# Autodesk Inventor assembly: Lift.03.01.00.00
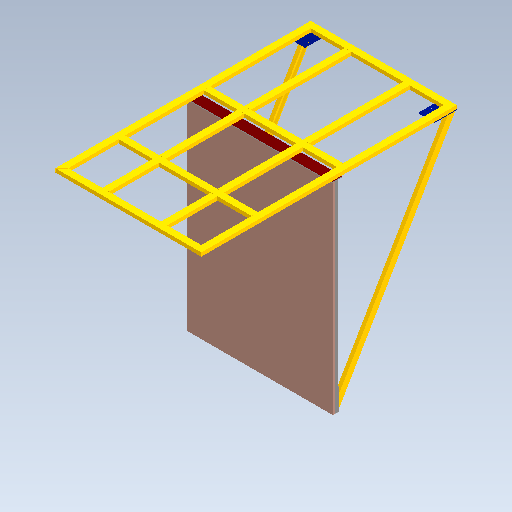
[picture p0: Inventor's stored thumbnail of the model, 512x512]
Saved by Autodesk Inventor 2021 (Build 250183000, 183)
## iProperties
_SolveAssemblyDoc: Frame Generator Solve Assembly
_Version: 15.0.0
Created: 2020-09-20
Part Number: Lift.03.01.00.00
Document SubType Name: Assembly
Designer: Kostya
Author: Kostya
## Documents named in this file (8)
- C:\Lift\Lift.03.01.00.00.iam
- C:\Lift\Lift.03.01.02.00.ipt
- C:\Lift\Lift.03.01.00.00\Frame\Frame 1600622124454.iam
- C:\Lift\Lift.03.01.01.00.iam
- C:\Lift\Lift.03.01.00.03.ipt
- C:\Lift\Lift.03.01.00.02_MIR.ipt
- C:\Lift\Lift.03.01.00.05.ipt
- C:\Lift\Lift.03.01.00.06.ipt
## Components (9 placed, 7 different names)
1. Lift.03.01.02.00:1
2. Frame 1600622124454:1 [sub-assembly] — Заподлицо:4, Заподлицо:5, Заподлицо:6, Заподлицо:7, Заподлицо:8, Совмещение:5, Совмещение:6, Совмещение:7, Заподлицо:12, Совмещение:8, Совмещение:9, Совмещение:10, Заподлицо:15
3. Lift.03.01.01.00:1 [sub-assembly] — Совмещение:4, Заподлицо:10, Заподлицо:11, Совмещение:11, Совмещение:12, Заподлицо:16, Заподлицо:17
4. Lift.03.01.00.03:1 — Совмещение:4, Заподлицо:10, Совмещение:5, Заподлицо:11, Заподлицо:12
5. Lift.03.01.00.02_MIR:1 — Заподлицо:4, Заподлицо:5, Совмещение:7, Заподлицо:14
6. Lift.03.01.00.02_MIR:2 — Заподлицо:7, Заподлицо:8, Совмещение:6, Заподлицо:13
7. Lift.03.01.00.05:1 — Заподлицо:13, Совмещение:8, Совмещение:9
8. Lift.03.01.00.05:2 — Совмещение:10, Заподлицо:14, Заподлицо:15, Совмещение:11
9. Lift.03.01.00.06:1 — Совмещение:12, Заподлицо:16, Заподлицо:17
## Relationships (22: Flush 13, Mate 9)
- Заподлицо:4 [Flush]: Frame 1600622124454:1 ↔ Lift.03.01.00.02_MIR:1
- Заподлицо:5 [Flush]: Frame 1600622124454:1 ↔ Lift.03.01.00.02_MIR:1
- Заподлицо:6 [Flush] (-920 mm): Frame 1600622124454:1
- Заподлицо:7 [Flush]: Frame 1600622124454:1 ↔ Lift.03.01.00.02_MIR:2
- Заподлицо:8 [Flush]: Frame 1600622124454:1 ↔ Lift.03.01.00.02_MIR:2
- Совмещение:4 [Mate]: Lift.03.01.01.00:1 ↔ Lift.03.01.00.03:1
- Заподлицо:10 [Flush]: Lift.03.01.01.00:1 ↔ Lift.03.01.00.03:1
- Совмещение:5 [Mate]: Frame 1600622124454:1 ↔ Lift.03.01.00.03:1
- Совмещение:6 [Mate]: Frame 1600622124454:1 ↔ Lift.03.01.00.02_MIR:2
- Совмещение:7 [Mate]: Frame 1600622124454:1 ↔ Lift.03.01.00.02_MIR:1
- Заподлицо:13 [Flush]: Lift.03.01.00.02_MIR:2 ↔ Lift.03.01.00.05:1
- Заподлицо:11 [Flush]: Lift.03.01.01.00:1 ↔ Lift.03.01.00.03:1
- Заподлицо:12 [Flush]: Frame 1600622124454:1 ↔ Lift.03.01.00.03:1
- Совмещение:8 [Mate] (-30 mm): Frame 1600622124454:1 ↔ Lift.03.01.00.05:1
- Совмещение:9 [Mate] (-50 mm): Frame 1600622124454:1 ↔ Lift.03.01.00.05:1
- Совмещение:10 [Mate] (-50 mm): Frame 1600622124454:1 ↔ Lift.03.01.00.05:2
- Заподлицо:14 [Flush]: Lift.03.01.00.02_MIR:1 ↔ Lift.03.01.00.05:2
- Заподлицо:15 [Flush] (30 mm): Frame 1600622124454:1 ↔ Lift.03.01.00.05:2
- Совмещение:11 [Mate]: Lift.03.01.01.00:1 ↔ Lift.03.01.00.05:2
- Совмещение:12 [Mate]: Lift.03.01.01.00:1 ↔ Lift.03.01.00.06:1
- Заподлицо:16 [Flush]: Lift.03.01.01.00:1 ↔ Lift.03.01.00.06:1
- Заподлицо:17 [Flush]: Lift.03.01.01.00:1 ↔ Lift.03.01.00.06:1
